# Autodesk Inventor assembly: leg
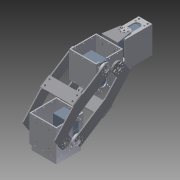
[picture p0: Inventor's stored thumbnail of the model, 180x180]
Saved by Autodesk Inventor 2013 (Build 170138000, 138)
## iProperties
Created: 2014-03-10
Part Number: leg
Document SubType Name: Assembly
Designer: ko
Author: ko
## Documents named in this file (12)
- C:\Users\andou\Documents\GitHub\Robotics-Project\design\RoboticsProject\project_4\Leg.iam
- C:\Users\andou\Documents\GitHub\Robotics-Project\design\RoboticsProject\project_4\Right_Parallel_Case.ipt
- C:\Users\andou\Documents\GitHub\Robotics-Project\design\RoboticsProject\project_4\Serial_Case.ipt
- C:\Users\andou\Documents\GitHub\Robotics-Project\design\RoboticsProject\project_4\Generic Parts\KRS-2500_serios.ipt
- C:\Users\andou\Documents\GitHub\Robotics-Project\design\RoboticsProject\project_4\Dual_Link_Flame(left).ipt
- C:\Users\andou\Documents\GitHub\Robotics-Project\design\RoboticsProject\project_4\Bracket.ipt
- C:\Users\andou\Documents\GitHub\Robotics-Project\design\RoboticsProject\project_4\Generic Parts\Low_Height_Horn.ipt
- C:\Users\andou\Documents\GitHub\Robotics-Project\design\RoboticsProject\project_4\Free-Horn.iam
- C:\Users\andou\Documents\GitHub\Robotics-Project\design\RoboticsProject\project_4\Parallel_Link_Supporter.ipt
- C:\Users\andou\Documents\GitHub\Robotics-Project\design\RoboticsProject\project_4\Sole_Spacer.ipt
- C:\Users\andou\Documents\GitHub\Robotics-Project\design\RoboticsProject\project_4\Horn-Spacer.ipt
- C:\Users\andou\Documents\GitHub\Robotics-Project\design\RoboticsProject\project_4\Dual_Link_Flame(right).ipt
## Components (26 placed, 11 different names)
1. Right_Parallel_Case:1 — 挿入:1, 挿入:2, 挿入:5, 挿入:6, 挿入:26, 挿入:27, 挿入:80
2. Right_Parallel_Case:2 — 挿入:43, 挿入:44, 挿入:46, 挿入:47, 挿入:63, 挿入:64, 挿入:79
3. Serial_Case:1 — 挿入:3, 挿入:4, 挿入:25
4. KRS-2500_serios:1 — 挿入:3, 挿入:4, 挿入:9
5. KRS-2500_serios:2 — 挿入:5, 挿入:6, 挿入:17
6. KRS-2500_serios:3 — 挿入:18, 挿入:43, 挿入:44
7. Dual_Link_Flame(left):3 — 挿入:32, 挿入:33, 挿入:55, 挿入:56, 挿入:65
8. Dual_Link_Flame(left):4 — 挿入:41, 挿入:54, 挿入:58, 挿入:66
9. Bracket:1 — 挿入:1, 挿入:2, 挿入:60, 挿入:61
10. Low_Height_Horn:1 — 挿入:9, 挿入:60
11. Low_Height_Horn:2 — 挿入:17, 挿入:68, 挿入:74
12. Low_Height_Horn:3 — 挿入:18, 挿入:67, 挿入:71
13. Free-Horn:1 [sub-assembly] — 挿入:25, 挿入:61
14. Free-Horn:2 [sub-assembly] — 挿入:26, 挿入:32, 挿入:33
15. Free-Horn:4 [sub-assembly] — 挿入:27, 挿入:41
16. Free-Horn:5 [sub-assembly] — 挿入:46, 挿入:54
17. Free-Horn:7 [sub-assembly] — 挿入:47, 挿入:55
18. Parallel_Link_Supporter:1 — 挿入:56, 挿入:65, 挿入:75, 挿入:76
19. Parallel_Link_Supporter:2 — 挿入:58, 挿入:66, 挿入:77, 挿入:78
20. Sole_Spacer:1 — 挿入:63, 挿入:64
21. Horn-Spacer:1 — 挿入:67
22. Horn-Spacer:2 — 挿入:68
23. Dual_Link_Flame(right):1 — 挿入:74, 挿入:75, 挿入:76, 挿入:81
24. Dual_Link_Flame(right):2 — 挿入:71, 挿入:77, 挿入:78, 挿入:82
25. Free-Horn:8 [sub-assembly] — 挿入:79, 挿入:81
26. Free-Horn:9 [sub-assembly] — 挿入:80, 挿入:82
## Relationships (41: Insert 41)
- 挿入:1 [Insert]: Right_Parallel_Case:1 ↔ Bracket:1
- 挿入:2 [Insert]: Right_Parallel_Case:1 ↔ Bracket:1
- 挿入:3 [Insert]: Serial_Case:1 ↔ KRS-2500_serios:1
- 挿入:4 [Insert]: Serial_Case:1 ↔ KRS-2500_serios:1
- 挿入:5 [Insert]: Right_Parallel_Case:1 ↔ KRS-2500_serios:2
- 挿入:6 [Insert]: Right_Parallel_Case:1 ↔ KRS-2500_serios:2
- 挿入:9 [Insert]: KRS-2500_serios:1 ↔ Low_Height_Horn:1
- 挿入:17 [Insert]: KRS-2500_serios:2 ↔ Low_Height_Horn:2
- 挿入:18 [Insert]: KRS-2500_serios:3 ↔ Low_Height_Horn:3
- 挿入:25 [Insert]: Serial_Case:1 ↔ Free-Horn:1
- 挿入:26 [Insert]: Right_Parallel_Case:1 ↔ Free-Horn:2
- 挿入:27 [Insert]: Right_Parallel_Case:1 ↔ Free-Horn:4
- 挿入:32 [Insert]: Dual_Link_Flame(left):3 ↔ Free-Horn:2
- 挿入:33 [Insert]: Dual_Link_Flame(left):3 ↔ Free-Horn:2
- 挿入:41 [Insert]: Dual_Link_Flame(left):4 ↔ Free-Horn:4
- 挿入:43 [Insert]: Right_Parallel_Case:2 ↔ KRS-2500_serios:3
- 挿入:44 [Insert]: Right_Parallel_Case:2 ↔ KRS-2500_serios:3
- 挿入:46 [Insert]: Right_Parallel_Case:2 ↔ Free-Horn:5
- 挿入:47 [Insert]: Right_Parallel_Case:2 ↔ Free-Horn:7
- 挿入:54 [Insert]: Dual_Link_Flame(left):4 ↔ Free-Horn:5
- 挿入:55 [Insert]: Dual_Link_Flame(left):3 ↔ Free-Horn:7
- 挿入:56 [Insert]: Dual_Link_Flame(left):3 ↔ Parallel_Link_Supporter:1
- 挿入:58 [Insert]: Dual_Link_Flame(left):4 ↔ Parallel_Link_Supporter:2
- 挿入:60 [Insert]: Bracket:1 ↔ Low_Height_Horn:1
- 挿入:61 [Insert]: Bracket:1 ↔ Free-Horn:1
- 挿入:63 [Insert]: Right_Parallel_Case:2 ↔ Sole_Spacer:1
- 挿入:64 [Insert]: Right_Parallel_Case:2 ↔ Sole_Spacer:1
- 挿入:65 [Insert]: Dual_Link_Flame(left):3 ↔ Parallel_Link_Supporter:1
- 挿入:66 [Insert]: Dual_Link_Flame(left):4 ↔ Parallel_Link_Supporter:2
- 挿入:67 [Insert]: Low_Height_Horn:3 ↔ Horn-Spacer:1
- 挿入:68 [Insert]: Low_Height_Horn:2 ↔ Horn-Spacer:2
- 挿入:71 [Insert]: Low_Height_Horn:3 ↔ Dual_Link_Flame(right):2
- 挿入:74 [Insert]: Low_Height_Horn:2 ↔ Dual_Link_Flame(right):1
- 挿入:75 [Insert]: Parallel_Link_Supporter:1 ↔ Dual_Link_Flame(right):1
- 挿入:76 [Insert]: Parallel_Link_Supporter:1 ↔ Dual_Link_Flame(right):1
- 挿入:77 [Insert]: Parallel_Link_Supporter:2 ↔ Dual_Link_Flame(right):2
- 挿入:78 [Insert]: Parallel_Link_Supporter:2 ↔ Dual_Link_Flame(right):2
- 挿入:79 [Insert]: Right_Parallel_Case:2 ↔ Free-Horn:8
- 挿入:80 [Insert]: Right_Parallel_Case:1 ↔ Free-Horn:9
- 挿入:81 [Insert]: Dual_Link_Flame(right):1 ↔ Free-Horn:8
- 挿入:82 [Insert]: Dual_Link_Flame(right):2 ↔ Free-Horn:9
